# Autodesk Inventor assembly: VersaBlock Pair
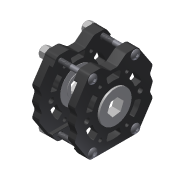
[picture p0: Inventor's stored thumbnail of the model, 180x180]
Saved by Autodesk Inventor 2013 (Build 170138000, 138)
## iProperties
Created: 2013-12-19
Part Number: VersaBlock Pair
Document SubType Name: Assembly
Designer: Niemitalo_Dan
Mass: 165.6 g
Surface Area: 284.613 cm^2
Volume: 48.4405 cm^3
Density: 3.41863 g/cm^3
Author: Niemitalo_Dan
## Documents named in this file (5)
- H:\Nemo\Documents\Robotics\CAD Files\COTS Parts\VersaFrame\VersaBlock Pair.iam
- H:\Nemo\Documents\Robotics\CAD Files\COTS Parts\Bearings - VexPro\Flanged Bearing - 0.5in Hex ID x 1.125in OD.ipt
- H:\Nemo\Documents\Robotics\CAD Files\COTS Parts\VersaFrame\VersaBlock.ipt
- H:\Nemo\Documents\Robotics\CAD Files\COTS Parts\Fasteners\8-32 locknut.ipt
- H:\Nemo\Documents\Robotics\CAD Files\COTS Parts\Fasteners\8-32 BHCS x1750.ipt
## Components (12 placed, 4 different names)
1. Flanged Bearing - 0.5in Hex ID x 1.125in OD:1 — Insert:2
2. Flanged Bearing - 0.5in Hex ID x 1.125in OD:2 — Insert:1
3. VersaBlock:1 — Flush:1, Flush:2, Flush:3, Insert:2, Insert:3, Insert:4, Insert:5, Insert:6
4. VersaBlock:2 — Mate:1, Flush:2, Mate:2, Insert:1, Insert:7, Insert:8, Insert:9, Insert:10
5. 8-32 locknut:1 — Insert:3
6. 8-32 locknut:2 — Insert:4
7. 8-32 locknut:3 — Insert:5
8. 8-32 locknut:4 — Insert:6
9. 8-32 BHCS x1750:1 — Insert:7
10. 8-32 BHCS x1750:2 — Insert:8
11. 8-32 BHCS x1750:3 — Insert:9
12. 8-32 BHCS x1750:4 — Insert:10
## Relationships (16: Insert 10, Flush 4, Mate 2)
- Flush:1 (12.7 mm): VersaBlock:1
- Flush:2: VersaBlock:1
- Flush:3: VersaBlock:1
- Mate:1: VersaBlock:2
- Flush:2: VersaBlock:2
- Mate:2 (12.7 mm): VersaBlock:2
- Insert:1: Flanged Bearing - 0.5in Hex ID x 1.125in OD:2 ↔ VersaBlock:2
- Insert:2: Flanged Bearing - 0.5in Hex ID x 1.125in OD:1 ↔ VersaBlock:1
- Insert:3: VersaBlock:1 ↔ 8-32 locknut:1
- Insert:4: VersaBlock:1 ↔ 8-32 locknut:2
- Insert:5: VersaBlock:1 ↔ 8-32 locknut:3
- Insert:6: VersaBlock:1 ↔ 8-32 locknut:4
- Insert:7: VersaBlock:2 ↔ 8-32 BHCS x1750:1
- Insert:8: VersaBlock:2 ↔ 8-32 BHCS x1750:2
- Insert:9: VersaBlock:2 ↔ 8-32 BHCS x1750:3
- Insert:10: VersaBlock:2 ↔ 8-32 BHCS x1750:4
